# Autodesk Inventor assembly: wheel
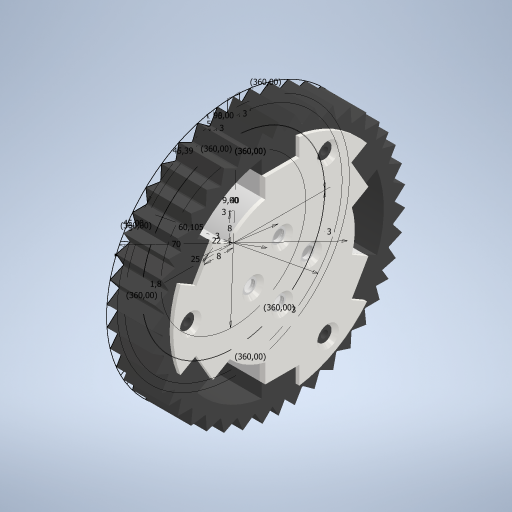
[picture p0: Inventor's stored thumbnail of the model, 512x512]
Saved by Autodesk Inventor 2023 (Build 270158000, 158)
## iProperties
Created: 2026-02-21
Part Number: wheel
Document SubType Name: Assembly
Designer: garin
Author: garin
## Documents named in this file (6)
- C:\Users\garin\OneDrive\Документы\maze\version1\wheel.iam
- C:\Users\garin\OneDrive\Документы\maze\version1\tire.ipt
- C:\Users\garin\OneDrive\Документы\maze\version1\wheel_mold.ipt
- C:\Users\garin\OneDrive\Документы\maze\version1\inside_part_wheel.ipt
- C:\Users\garin\OneDrive\Документы\maze\version1\top_part_wheel.ipt
- C:\Users\garin\OneDrive\Документы\maze\version1\low_part_wheel.ipt
## Components (5 placed, 5 different names)
1. tire:1 — Заподлицо:1, Заподлицо:2, Заподлицо:3, С поворотом:2, С поворотом:3
2. inside_part_wheel:1 — Заподлицо:2
3. top_part_wheel:1 — Заподлицо:3, С поворотом:3
4. low_part_wheel:1 — С поворотом:2
5. wheel_mold:1 — Заподлицо:1
## Relationships (5: Flush 3, RevoluteJoint 2)
- Заподлицо:1 [Flush]: tire:1 ↔ wheel_mold:1
- Заподлицо:2 [Flush]: tire:1 ↔ inside_part_wheel:1
- Заподлицо:3 [Flush]: tire:1 ↔ top_part_wheel:1
- С поворотом:2 [RevoluteJoint]: tire:1 ↔ low_part_wheel:1
- С поворотом:3 [RevoluteJoint]: tire:1 ↔ top_part_wheel:1
